# Autodesk Inventor assembly: assembly
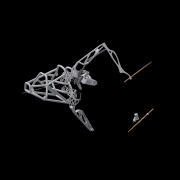
[picture p0: Inventor's stored thumbnail of the model, 180x180]
Saved by Autodesk Inventor 2020 (Build 240168000, 168)
## iProperties
Created: 2020-03-24
Part Number: assembly
Document SubType Name: Assembly
Designer: valer
Author: valer
## Documents named in this file (23)
- C:\Users\valer\Desktop\drummingrobot\src\Robot.iam
- C:\Users\valer\Desktop\drummingrobot\src\Chest.ipt
- C:\Users\valer\Desktop\drummingrobot\src\HeadScaled.ipt
- C:\Users\valer\Desktop\drummingrobot\src\UpperArmServoDynamixelXM430-W350-T.ipt
- C:\Users\valer\Desktop\drummingrobot\src\UpperArm.ipt
- C:\Users\valer\Desktop\drummingrobot\src\UpperArmBracket.ipt
- C:\Users\valer\Desktop\drummingrobot\src\UpperArmMount.ipt
- C:\Users\valer\Desktop\drummingrobot\src\external\ShoulderConnectingRod.ipt
- C:\Users\valer\Desktop\drummingrobot\src\Forearm.ipt
- C:\Users\valer\Desktop\drummingrobot\src\external\Drumstick.ipt
- C:\Users\valer\Desktop\drummingrobot\src\external\ForearmShaftCollar.ipt
- C:\Users\valer\Desktop\drummingrobot\src\external\RodEndFixed.ipt
- C:\Users\valer\Desktop\drummingrobot\src\ShoulderBracket.ipt
- C:\Users\valer\Desktop\drummingrobot\src\ChestShoulderBracket.ipt
- C:\Users\valer\Desktop\drummingrobot\src\ChestShoulderBracketMirror.ipt
- C:\Users\valer\Desktop\drummingrobot\src\external\PullSolenoid.ipt
- C:\Users\valer\Desktop\drummingrobot\src\external\PushSolenoid.ipt
- C:\Users\valer\Desktop\drummingrobot\src\external\UpperArmActuatorBody.ipt
- C:\Users\valer\Desktop\drummingrobot\src\external\UpperArmActuatorShaft.ipt
- C:\Users\valer\Desktop\drummingrobot\src\external\ForearmActuatorBody.ipt
- C:\Users\valer\Desktop\drummingrobot\src\external\ForearmActuatorShaft.ipt
- C:\Users\valer\Desktop\drummingrobot\src\external\Drums.ipt
- C:\Users\valer\Desktop\drummingrobot\src\ForearmActuatorConnector.ipt
## Components (57 placed, 21 different names)
1. Chest:1 — Angle:1, Angle:6, Mate:117, Mate:118, Mate:119, Mate:120, Mate:121, Mate:122, Mate:130, Mate:131, Mate:132, Mate:133, Mate:134, Mate:157
2. HeadScaled:1 — Angle:6
3. UpperArmServoDynamixelXM430-W350-T:1 — Angle:1, Mate:10, Mate:11, Mate:116, Angle:7, Mate:164
4. UpperArmBracket:1 — Mate:6, Mate:8, Mate:25, Mate:235
5. UpperArmMount:1 — Mate:6, Mate:7, Mate:8, Mate:10, Mate:11, Mate:25, Mate:78, Angle:9
6. UpperArmBracket:2 — Mate:7, Mate:78, Mate:226, Mate:235, Mate:237
7. ChestConnectingRod:1 — Mate:88, Mate:89, Mate:105
8. ChestConnectingRod:2 — Mate:86, Mate:87, Mate:104
9. ChestConnectingRod:3 — Mate:84, Mate:85, Mate:98
10. ChestConnectingRod:4 — Mate:82, Mate:83, Mate:97
11. Drumstick:1 — Mate:79, Flush:3
12. ShaftCollar1/2:1 — Mate:79, Flush:3, Mate:236, Flush:18
13. RodEnd1/4-1/4-1:1 — Mate:82, Mate:115
14. RodEnd1/4-1/4-1:2 — Mate:83, Mate:97, Mate:123, Mate:125
15. RodEnd1/4-1/4-1:3 — Mate:84, Mate:114
16. RodEnd1/4-1/4-1:4 — Mate:85, Mate:98, Mate:124, Mate:142
17. RodEnd1/4-1/4-1:5 — Mate:86, Mate:110
18. RodEnd1/4-1/4-1:6 — Mate:87, Mate:104, Mate:126, Mate:129
19. RodEnd1/4-1/4-1:7 — Mate:88, Mate:109
20. RodEnd1/4-1/4-1:8 — Mate:89, Mate:105, Mate:127, Mate:128
21. ShoulderBracket:2 — Mate:109, Mate:110, Flush:6, Mate:116, Angle:7, Flush:9, Mate:164, Flush:14
22. ShoulderBracket:3 — Flush:6, Mate:114, Mate:115, Flush:8, Flush:14
23. ChestShoulderBracket:1 — Mate:120, Mate:121, Mate:122, Mate:123, Mate:124, Flush:8, Mate:125, Mate:142
24. ChestShoulderBracketMirror:1 — Mate:117, Mate:118, Mate:119, Mate:126, Mate:127, Flush:9, Mate:128, Mate:129
25. ChestShoulderBracket:2 — Mate:130, Mate:131, Mate:157, Mate:160, Mate:162, Mate:213, Mate:214
26. ShoulderBracket:4 — Mate:144, Mate:145, Mate:147, Mate:196, Flush:15
27. ShoulderBracket:5 — Mate:159, Mate:199, Mate:209, Mate:211, Mate:212, Flush:15
28. ChestShoulderBracketMirror:2 — Mate:132, Mate:133, Mate:134, Mate:141, Mate:146, Mate:148, Mate:149
29. ChestConnectingRod:5
30. ChestConnectingRod:6
31. RodEnd1/4-1/4-1:9 — Mate:144, Mate:145
32. RodEnd1/4-1/4-1:10 — Mate:148, Mate:149
33. RodEnd1/4-1/4-1:11 — Mate:147
34. RodEnd1/4-1/4-1:12 — Mate:141, Mate:146
35. ChestConnectingRod:7
36. ChestConnectingRod:8
37. RodEnd1/4-1/4-1:13 — Mate:211, Mate:212
38. RodEnd1/4-1/4-1:14 — Mate:162, Mate:214
39. RodEnd1/4-1/4-1:15 — Mate:159, Mate:209
40. RodEnd1/4-1/4-1:16 — Mate:160, Mate:213
41. UpperArmServoDynamixelXM430-W350-T:2 — Mate:196, Mate:199
42. UpperArm:2
43. UpperArmBracket:3
44. UpperArmMount:2 — Angle:9
45. UpperArmBracket:4
46. Drumstick:2 — Mate:181
47. ShaftCollar1/2:2 — Mate:181
48. PullSolenoid:1
49. PushSolenoid:1
50. FA-35-S-12-1:1 — Mate:182, Mate:183
51. Forearm:1 — Flush:17, Mate:227, Mate:236, Flush:18, Mate:239
52. FA-35-S-12-1:2 — Mate:182, Mate:183, Mate:238, Flush:20
53. ForearmActuatorBody:1 — Mate:231, Mate:232, Mate:234, Flush:19
54. Drums:1 — Flush:13
55. ForearmActuatorShaft:3 — Flush:17, Mate:231, Mate:232, Mate:241, Mate:242
56. UpperArm:3 — Mate:226, Mate:227, Mate:234, Mate:237, Mate:238, Flush:19, Flush:20
57. ForearmActuatorConnector:1 — Mate:239, Mate:241, Mate:242
## Relationships (117: Mate 100, Flush 13, Angle 4)
- Angle:1 (0 deg): Chest:1 ↔ UpperArmServoDynamixelXM430-W350-T:1
- Mate:6: UpperArmBracket:1 ↔ UpperArmMount:1
- Mate:7: UpperArmMount:1 ↔ UpperArmBracket:2
- Mate:8: UpperArmBracket:1 ↔ UpperArmMount:1
- Mate:10: UpperArmServoDynamixelXM430-W350-T:1 ↔ UpperArmMount:1
- Mate:11: UpperArmServoDynamixelXM430-W350-T:1 ↔ UpperArmMount:1
- Mate:25 (12.7 mm): UpperArmBracket:1 ↔ UpperArmMount:1
- Angle:6 (0 deg): Chest:1 ↔ HeadScaled:1
- Mate:78: UpperArmMount:1 ↔ UpperArmBracket:2
- Mate:79: Drumstick:1 ↔ ShaftCollar1/2:1
- Flush:3 (304.8 mm): Drumstick:1 ↔ ShaftCollar1/2:1
- Mate:82: ChestConnectingRod:4 ↔ RodEnd1/4-1/4-1:1
- Mate:83: ChestConnectingRod:4 ↔ RodEnd1/4-1/4-1:2
- Mate:84: ChestConnectingRod:3 ↔ RodEnd1/4-1/4-1:3
- Mate:85: ChestConnectingRod:3 ↔ RodEnd1/4-1/4-1:4
- Mate:86: ChestConnectingRod:2 ↔ RodEnd1/4-1/4-1:5
- Mate:87: ChestConnectingRod:2 ↔ RodEnd1/4-1/4-1:6
- Mate:88: ChestConnectingRod:1 ↔ RodEnd1/4-1/4-1:7
- Mate:89: ChestConnectingRod:1 ↔ RodEnd1/4-1/4-1:8
- Mate:97 (-25.4 mm): ChestConnectingRod:4 ↔ RodEnd1/4-1/4-1:2
- Mate:98 (-25.4 mm): ChestConnectingRod:3 ↔ RodEnd1/4-1/4-1:4
- Mate:104 (-25.4 mm): ChestConnectingRod:2 ↔ RodEnd1/4-1/4-1:6
- Mate:105 (-25.4 mm): ChestConnectingRod:1 ↔ RodEnd1/4-1/4-1:8
- Mate:109: RodEnd1/4-1/4-1:7 ↔ ShoulderBracket:2
- Mate:110: RodEnd1/4-1/4-1:5 ↔ ShoulderBracket:2
- Flush:6: ShoulderBracket:2 ↔ ShoulderBracket:3
- Mate:114: RodEnd1/4-1/4-1:3 ↔ ShoulderBracket:3
- Mate:115: RodEnd1/4-1/4-1:1 ↔ ShoulderBracket:3
- Mate:116: UpperArmServoDynamixelXM430-W350-T:1 ↔ ShoulderBracket:2
- Angle:7 (0 deg): UpperArmServoDynamixelXM430-W350-T:1 ↔ ShoulderBracket:2
- Mate:117: Chest:1 ↔ ChestShoulderBracketMirror:1
- Mate:118: Chest:1 ↔ ChestShoulderBracketMirror:1
- Mate:119: Chest:1 ↔ ChestShoulderBracketMirror:1
- Mate:120: Chest:1 ↔ ChestShoulderBracket:1
- Mate:121: Chest:1 ↔ ChestShoulderBracket:1
- Mate:122: Chest:1 ↔ ChestShoulderBracket:1
- Mate:123: RodEnd1/4-1/4-1:2 ↔ ChestShoulderBracket:1
- Mate:124: RodEnd1/4-1/4-1:4 ↔ ChestShoulderBracket:1
- Flush:8: ShoulderBracket:3 ↔ ChestShoulderBracket:1
- Mate:125: RodEnd1/4-1/4-1:2 ↔ ChestShoulderBracket:1
- Mate:126: RodEnd1/4-1/4-1:6 ↔ ChestShoulderBracketMirror:1
- Mate:127: RodEnd1/4-1/4-1:8 ↔ ChestShoulderBracketMirror:1
- Flush:9: ShoulderBracket:2 ↔ ChestShoulderBracketMirror:1
- Mate:128: RodEnd1/4-1/4-1:8 ↔ ChestShoulderBracketMirror:1
- Mate:129: RodEnd1/4-1/4-1:6 ↔ ChestShoulderBracketMirror:1
- Mate:130: Chest:1 ↔ ChestShoulderBracket:2
- Mate:131: Chest:1 ↔ ChestShoulderBracket:2
- [Flush]: ShoulderBracket:4 ↔ ShoulderBracket:5
- Mate:132: Chest:1 ↔ ChestShoulderBracketMirror:2
- Mate:133: Chest:1 ↔ ChestShoulderBracketMirror:2
- Mate:134: Chest:1 ↔ ChestShoulderBracketMirror:2
- [Mate]: ChestConnectingRod:6 ↔ RodEnd1/4-1/4-1:9
- [Mate]: ChestConnectingRod:6 ↔ RodEnd1/4-1/4-1:10
- [Mate]: ChestConnectingRod:5 ↔ RodEnd1/4-1/4-1:11
- [Mate]: ChestConnectingRod:5 ↔ RodEnd1/4-1/4-1:12
- [Mate] (-25.4 mm): ChestConnectingRod:6 ↔ RodEnd1/4-1/4-1:10
- [Mate] (-25.4 mm): ChestConnectingRod:5 ↔ RodEnd1/4-1/4-1:12
- Mate:141: ChestShoulderBracketMirror:2 ↔ RodEnd1/4-1/4-1:12
- Mate:142: RodEnd1/4-1/4-1:4 ↔ ChestShoulderBracket:1
- Mate:144: ShoulderBracket:4 ↔ RodEnd1/4-1/4-1:9
- Mate:145: ShoulderBracket:4 ↔ RodEnd1/4-1/4-1:9
- Mate:146: ChestShoulderBracketMirror:2 ↔ RodEnd1/4-1/4-1:12
- Mate:147: ShoulderBracket:4 ↔ RodEnd1/4-1/4-1:11
- Mate:148: ChestShoulderBracketMirror:2 ↔ RodEnd1/4-1/4-1:10
- Mate:149: ChestShoulderBracketMirror:2 ↔ RodEnd1/4-1/4-1:10
- [Mate]: ChestConnectingRod:8 ↔ RodEnd1/4-1/4-1:13
- [Mate]: ChestConnectingRod:8 ↔ RodEnd1/4-1/4-1:14
- [Mate]: ChestConnectingRod:7 ↔ RodEnd1/4-1/4-1:15
- [Mate]: ChestConnectingRod:7 ↔ RodEnd1/4-1/4-1:16
- [Mate] (-25.4 mm): ChestConnectingRod:8 ↔ RodEnd1/4-1/4-1:14
- [Mate] (-25.4 mm): ChestConnectingRod:7 ↔ RodEnd1/4-1/4-1:16
- Mate:157: Chest:1 ↔ ChestShoulderBracket:2
- Mate:159: ShoulderBracket:5 ↔ RodEnd1/4-1/4-1:15
- Mate:160: ChestShoulderBracket:2 ↔ RodEnd1/4-1/4-1:16
- Mate:162: ChestShoulderBracket:2 ↔ RodEnd1/4-1/4-1:14
- Mate:164 (12.7 mm): UpperArmServoDynamixelXM430-W350-T:1 ↔ ShoulderBracket:2
- [Mate]: UpperArm:2 ↔ UpperArmBracket:3
- [Mate]: UpperArm:2 ↔ UpperArmBracket:4
- [Mate]: UpperArm:2 ↔ UpperArmBracket:4
- [Mate]: UpperArmBracket:3 ↔ UpperArmMount:2
- [Mate]: UpperArmMount:2 ↔ UpperArmBracket:4
- [Mate]: UpperArmBracket:3 ↔ UpperArmMount:2
- [Mate]: UpperArmServoDynamixelXM430-W350-T:2 ↔ UpperArmMount:2
- [Mate]: UpperArmServoDynamixelXM430-W350-T:2 ↔ UpperArmMount:2
- [Mate] (12.7 mm): UpperArmBracket:3 ↔ UpperArmMount:2
- [Mate]: UpperArmMount:2 ↔ UpperArmBracket:4
- [Flush] (304.8 mm): Drumstick:2 ↔ ShaftCollar1/2:2
- Mate:181: Drumstick:2 ↔ ShaftCollar1/2:2
- Mate:182: FA-35-S-12-1:1 ↔ FA-35-S-12-1:2
- Mate:183: FA-35-S-12-1:1 ↔ FA-35-S-12-1:2
- Angle:9 (169.89 deg): UpperArmMount:1 ↔ UpperArmMount:2
- Mate:196: ShoulderBracket:4 ↔ UpperArmServoDynamixelXM430-W350-T:2
- Mate:199 (12.7 mm): ShoulderBracket:5 ↔ UpperArmServoDynamixelXM430-W350-T:2
- Flush:13 (508 mm): Drums:1
- Flush:14: ShoulderBracket:2 ↔ ShoulderBracket:3
- Mate:209: ShoulderBracket:5 ↔ RodEnd1/4-1/4-1:15
- Mate:211: ShoulderBracket:5 ↔ RodEnd1/4-1/4-1:13
- Mate:212: ShoulderBracket:5 ↔ RodEnd1/4-1/4-1:13
- Mate:213: ChestShoulderBracket:2 ↔ RodEnd1/4-1/4-1:16
- Mate:214: ChestShoulderBracket:2 ↔ RodEnd1/4-1/4-1:14
- Flush:15: ShoulderBracket:4 ↔ ShoulderBracket:5
- Flush:17: Forearm:1 ↔ ForearmActuatorShaft:3
- Mate:226: UpperArmBracket:2 ↔ UpperArm:3
- Mate:227: Forearm:1 ↔ UpperArm:3
- Mate:231: ForearmActuatorBody:1 ↔ ForearmActuatorShaft:3
- Mate:232: ForearmActuatorBody:1 ↔ ForearmActuatorShaft:3
- Mate:234: ForearmActuatorBody:1 ↔ UpperArm:3
- Mate:235: UpperArmBracket:1 ↔ UpperArmBracket:2
- Mate:236: ShaftCollar1/2:1 ↔ Forearm:1
- Flush:18 (12.7 mm): ShaftCollar1/2:1 ↔ Forearm:1
- Mate:237: UpperArmBracket:2 ↔ UpperArm:3
- Mate:238: FA-35-S-12-1:2 ↔ UpperArm:3
- Flush:19: ForearmActuatorBody:1 ↔ UpperArm:3
- Flush:20: FA-35-S-12-1:2 ↔ UpperArm:3
- Mate:239: Forearm:1 ↔ ForearmActuatorConnector:1
- Mate:241: ForearmActuatorShaft:3 ↔ ForearmActuatorConnector:1
- Mate:242: ForearmActuatorShaft:3 ↔ ForearmActuatorConnector:1
## Named parameters: d236_d209 = 0 mm, d244_d149 = 0 mm, d245_d150 = 0 mm, d246_d151 = 0 mm, d247_d152 = 0 mm, d248_d197 = -25.4 mm, d249_d198 = -25.4 mm, d259_d145 = 0 mm, d260_d146 = 0 mm, d261_d147 = 0 mm, d262_d148 = 0 mm, d263_d190 = -25.4 mm, d264_d191 = -25.4 mm, d274_d140 = 0 mm, d276_d142 = 304.8 mm, d278_d53 = 0 mm, d279_d54 = 0 mm, d280_d55 = 0 mm, d281_d56 = 0 mm, d282_d57 = 0 mm, d283_d58 = 0 mm, d284_d60 = 0 mm, d285_d61 = 0 mm, d286_d80 = 12.7 mm
